# Autodesk Inventor assembly: attachementOnExtresion
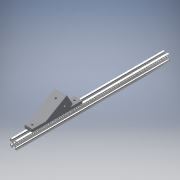
[picture p0: Inventor's stored thumbnail of the model, 180x180]
Saved by Autodesk Inventor 2019.3 (Build 233278000, 278)
## iProperties
Created: 2019-02-15
Part Number: attachementOnExtresion
Document SubType Name: Assembly
Designer: steele
Author: steele
## Documents named in this file (3)
- C:\git\CAD-Development\robSteele\RevRoboticsExtrusionAttachements\attachementOnExtresion.iam
- C:\git\CAD-Development\robSteele\RevRoboticsExtrusionAttachements\RevRobotics20inchExtrusion.ipt
- C:\git\CAD-Development\robSteele\RevRoboticsExtrusionAttachements\30DegreeAttachementV03.ipt
## Components (2 placed, 2 different names)
1. RevRobotics20inchExtrusion:1
2. 30DegreeAttachementV03:1
## Relationships (3: Mate 2, Flush 1)
- [Mate]: RevRobotics20inchExtrusion:1 ↔ 30DegreeAttachementV03:1
- [Mate]: RevRobotics20inchExtrusion:1 ↔ 30DegreeAttachementV03:1
- [Flush] (-50.8 mm): RevRobotics20inchExtrusion:1 ↔ 30DegreeAttachementV03:1
